# Autodesk Inventor assembly: Frame V2
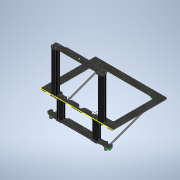
[picture p0: Inventor's stored thumbnail of the model, 180x180]
Saved by Autodesk Inventor 2020.3 (Build 243373010, 373A)
## iProperties
Created: 2019-06-17
Part Number: Frame V2
Document SubType Name: Assembly
Designer: pepd9
Author: pepd9
## Documents named in this file (13)
- D:\Designs\MK3PRO P1\FRAME\Frame V2.iam
- D:\Designs\MK3PRO P1\FRAME\FRONT PLATE P1.2.ipt
- D:\Designs\MK3PRO P1\FRAME\Long Extrusion.ipt
- D:\Designs\MK3PRO P1\COMPONENTS\90128A234_ZNC-PLTD ALLOY STL SCKT HEAD CAP SCREW.ipt
- D:\Designs\MK3PRO P1\FRAME\Short Extrusion.ipt
- D:\Designs\MK3PRO P1\FRAME\REAR PLATE P1.2.ipt
- D:\Designs\MK3PRO P1\FRAME\Angle Support Bottom Anchor.ipt
- D:\Designs\MK3PRO P1\FRAME\Angle Support Top Anchor.ipt
- D:\Designs\MK3PRO P1\COMPONENTS\WASHER_M10.ipt
- D:\Designs\MK3PRO P1\FRAME\Angle Support.ipt
- D:\Designs\MK3PRO P1\COMPONENTS\NUT_THIN_M10.ipt
- D:\Designs\MK3PRO P1\COMPONENTS\SHCS_M3_12.ipt
- D:\Designs\MK3PRO P1\FRAME\CENTER FRAME P2.0.ipt
## Components (85 placed, 12 different names)
1. CENTER FRAME P2.0:1 — Mate:1, Mate:2, Mate:3, Mate:4, Mate:5, Mate:6, Mate:7, Mate:8, Mate:9, Flush:1, Mate:23, Mate:24, Mate:25, Mate:28, Mate:37, Mate:38, Mate:39, Mate:40, Mate:41, Mate:42, Mate:43, Mate:44, Mate:45, Mate:46, Mate:47, Mate:48, Mate:49, Mate:50, Mate:51, Mate:52, Mate:53, Mate:54, Mate:55, Mate:56, Mate:57, Mate:58, Mate:59, Mate:60, Mate:61, Mate:62, Mate:63, Mate:64, Mate:65, Mate:66, Mate:96, Mate:97, Mate:98, Mate:99, Mate:100, Mate:101
2. Long Extrusion:1 — Mate:1, Mate:10, Mate:11, Mate:229
3. 90128A234_ZNC-PLTD ALLOY STL SCKT HEAD CAP SCREW:1 — Mate:2, Mate:3, Mate:10
4. 90128A234_ZNC-PLTD ALLOY STL SCKT HEAD CAP SCREW:2 — Mate:6, Mate:7
5. 90128A234_ZNC-PLTD ALLOY STL SCKT HEAD CAP SCREW:3 — Mate:5, Mate:8
6. 90128A234_ZNC-PLTD ALLOY STL SCKT HEAD CAP SCREW:4 — Mate:4, Mate:9, Mate:11
7. 90128A234_ZNC-PLTD ALLOY STL SCKT HEAD CAP SCREW:5 — Mate:231
8. 90128A234_ZNC-PLTD ALLOY STL SCKT HEAD CAP SCREW:6
9. 90128A234_ZNC-PLTD ALLOY STL SCKT HEAD CAP SCREW:7 — Mate:230
10. 90128A234_ZNC-PLTD ALLOY STL SCKT HEAD CAP SCREW:8
11. Long Extrusion:2 — Mate:25, Mate:28
12. 90128A234_ZNC-PLTD ALLOY STL SCKT HEAD CAP SCREW:9
13. 90128A234_ZNC-PLTD ALLOY STL SCKT HEAD CAP SCREW:10
14. 90128A234_ZNC-PLTD ALLOY STL SCKT HEAD CAP SCREW:11
15. 90128A234_ZNC-PLTD ALLOY STL SCKT HEAD CAP SCREW:12
16. 90128A234_ZNC-PLTD ALLOY STL SCKT HEAD CAP SCREW:13 — Mate:37, Mate:44
17. 90128A234_ZNC-PLTD ALLOY STL SCKT HEAD CAP SCREW:14 — Mate:38, Mate:42
18. 90128A234_ZNC-PLTD ALLOY STL SCKT HEAD CAP SCREW:15 — Mate:39, Mate:43
19. 90128A234_ZNC-PLTD ALLOY STL SCKT HEAD CAP SCREW:16 — Mate:40, Mate:41
20. Short Extrusion:1 — Mate:45, Mate:46, Mate:47
21. Short Extrusion:2 — Mate:48, Mate:49, Mate:50, Mate:67, Mate:68, Mate:69
22. 90128A234_ZNC-PLTD ALLOY STL SCKT HEAD CAP SCREW:17 — Mate:53, Mate:56
23. 90128A234_ZNC-PLTD ALLOY STL SCKT HEAD CAP SCREW:18 — Mate:54, Mate:58
24. 90128A234_ZNC-PLTD ALLOY STL SCKT HEAD CAP SCREW:19 — Mate:51, Mate:55
25. 90128A234_ZNC-PLTD ALLOY STL SCKT HEAD CAP SCREW:20 — Mate:52, Mate:57
26. 90128A234_ZNC-PLTD ALLOY STL SCKT HEAD CAP SCREW:21 — Mate:59, Mate:63
27. 90128A234_ZNC-PLTD ALLOY STL SCKT HEAD CAP SCREW:22 — Mate:60, Mate:64
28. 90128A234_ZNC-PLTD ALLOY STL SCKT HEAD CAP SCREW:23 — Mate:61, Mate:65
29. 90128A234_ZNC-PLTD ALLOY STL SCKT HEAD CAP SCREW:24 — Mate:62, Mate:66
30. REAR PLATE P1.2:1 — Mate:67, Mate:68, Mate:69, Mate:70, Mate:71, Mate:72, Mate:73, Mate:74, Mate:75, Mate:76, Mate:77, Mate:78, Mate:79, Mate:80, Mate:81, Mate:82, Mate:83, Mate:84, Mate:95, Mate:102, Mate:103
31. 90128A234_ZNC-PLTD ALLOY STL SCKT HEAD CAP SCREW:25 — Mate:70, Mate:83
32. 90128A234_ZNC-PLTD ALLOY STL SCKT HEAD CAP SCREW:26 — Mate:71, Mate:81
33. 90128A234_ZNC-PLTD ALLOY STL SCKT HEAD CAP SCREW:27 — Mate:73, Mate:84
34. 90128A234_ZNC-PLTD ALLOY STL SCKT HEAD CAP SCREW:28 — Mate:72, Mate:82
35. 90128A234_ZNC-PLTD ALLOY STL SCKT HEAD CAP SCREW:29 — Mate:76, Mate:78
36. 90128A234_ZNC-PLTD ALLOY STL SCKT HEAD CAP SCREW:30 — Mate:74, Mate:77
37. 90128A234_ZNC-PLTD ALLOY STL SCKT HEAD CAP SCREW:31 — Mate:75, Mate:79
38. 90128A234_ZNC-PLTD ALLOY STL SCKT HEAD CAP SCREW:32 — Mate:80, Mate:95
39. Angle Support Bottom Anchor:1 — Mate:102, Mate:104, Mate:106, Mate:107, Mate:108, Mate:109, Mate:168, Mate:169, Mate:170, Mate:171, Mate:172, Mate:173, Mate:174, Mate:175
40. Angle Support Bottom Anchor:2 — Mate:103, Mate:105, Mate:110, Mate:111, Mate:112, Mate:113, Mate:176, Mate:177, Mate:178, Mate:179, Mate:180, Mate:181, Mate:182, Mate:183
41. Angle Support Top Anchor:1 — Mate:96, Mate:98, Mate:99, Mate:104, Mate:114, Mate:115, Mate:116, Mate:117, Mate:122, Mate:156, Mate:157, Mate:158, Mate:159, Mate:184, Mate:185, Mate:186, Mate:187
42. Angle Support Top Anchor:2 — Mate:97, Mate:100, Mate:101, Mate:105, Mate:118, Mate:119, Mate:120, Mate:121, Mate:123, Mate:160, Mate:161, Mate:162, Mate:163, Mate:164, Mate:165, Mate:166, Mate:167
43. WASHER_M10:1 — Mate:116, Mate:117, Mate:138
44. WASHER_M10:2 — Mate:114, Mate:115, Mate:136
45. WASHER_M10:3 — Mate:119, Mate:120, Mate:130
46. WASHER_M10:4 — Mate:118, Mate:121, Mate:128
47. WASHER_M10:5 — Mate:110, Mate:111, Mate:149
48. WASHER_M10:6 — Mate:112, Mate:113, Mate:154
49. WASHER_M10:7 — Mate:106, Mate:107, Mate:141
50. WASHER_M10:8 — Mate:108, Mate:109, Mate:146
51. Angle Support:1 — Mate:122, Mate:132, Mate:133, Mate:134, Mate:135, Flush:2, Mate:140, Mate:142, Mate:144, Mate:145
52. Angle Support:2 — Mate:123, Mate:124, Mate:125, Mate:126, Mate:127, Flush:3, Mate:148, Mate:150, Mate:152, Mate:153
53. NUT_THIN_M10:1 — Mate:134, Mate:138, Mate:139
54. NUT_THIN_M10:2 — Mate:135, Mate:139
55. NUT_THIN_M10:3 — Mate:132, Mate:137, Flush:2
56. NUT_THIN_M10:4 — Mate:133, Mate:136, Mate:137
57. NUT_THIN_M10:5 — Mate:125, Mate:131, Flush:3
58. NUT_THIN_M10:6 — Mate:127, Mate:129
59. NUT_THIN_M10:7 — Mate:126, Mate:128, Mate:129
60. NUT_THIN_M10:8 — Mate:124, Mate:130, Mate:131
61. NUT_THIN_M10:9 — Mate:140, Mate:141, Mate:143
62. NUT_THIN_M10:10 — Mate:144, Mate:146, Mate:147
63. NUT_THIN_M10:11 — Mate:145, Mate:147
64. NUT_THIN_M10:12 — Mate:142, Mate:143
65. NUT_THIN_M10:13 — Mate:148, Mate:149, Mate:151
66. NUT_THIN_M10:14 — Mate:152, Mate:154, Mate:155
67. NUT_THIN_M10:15 — Mate:150, Mate:151
68. NUT_THIN_M10:16 — Mate:153, Mate:155, Flush:4
69. SHCS_M3_12:1 — Mate:171, Mate:175
70. SHCS_M3_12:2 — Mate:170, Mate:174
71. SHCS_M3_12:3 — Mate:169, Mate:172
72. SHCS_M3_12:4 — Mate:168, Mate:173
73. SHCS_M3_12:5 — Mate:179, Mate:180
74. SHCS_M3_12:6 — Mate:178, Mate:181
75. SHCS_M3_12:7 — Mate:177, Mate:183
76. SHCS_M3_12:8 — Mate:176, Mate:182
77. SHCS_M3_12:9 — Mate:156, Mate:184
78. SHCS_M3_12:10 — Mate:157, Mate:185
79. SHCS_M3_12:11 — Mate:158, Mate:186
80. SHCS_M3_12:12 — Mate:159, Mate:187
81. SHCS_M3_12:13 — Mate:163, Mate:167
82. SHCS_M3_12:14 — Mate:162, Mate:166
83. SHCS_M3_12:15 — Mate:161, Mate:165
84. SHCS_M3_12:16 — Mate:160, Mate:164
85. FRONT PLATE P1.2:1 — Mate:229, Mate:230, Mate:231
## Relationships (163: Mate 159, Flush 4)
- Mate:1: CENTER FRAME P2.0:1 ↔ Long Extrusion:1
- Mate:2: CENTER FRAME P2.0:1 ↔ 90128A234_ZNC-PLTD ALLOY STL SCKT HEAD CAP SCREW:1
- Mate:3: CENTER FRAME P2.0:1 ↔ 90128A234_ZNC-PLTD ALLOY STL SCKT HEAD CAP SCREW:1
- Mate:4: CENTER FRAME P2.0:1 ↔ 90128A234_ZNC-PLTD ALLOY STL SCKT HEAD CAP SCREW:4
- Mate:5: CENTER FRAME P2.0:1 ↔ 90128A234_ZNC-PLTD ALLOY STL SCKT HEAD CAP SCREW:3
- Mate:6: CENTER FRAME P2.0:1 ↔ 90128A234_ZNC-PLTD ALLOY STL SCKT HEAD CAP SCREW:2
- Mate:7: CENTER FRAME P2.0:1 ↔ 90128A234_ZNC-PLTD ALLOY STL SCKT HEAD CAP SCREW:2
- Mate:8: CENTER FRAME P2.0:1 ↔ 90128A234_ZNC-PLTD ALLOY STL SCKT HEAD CAP SCREW:3
- Mate:9: CENTER FRAME P2.0:1 ↔ 90128A234_ZNC-PLTD ALLOY STL SCKT HEAD CAP SCREW:4
- Mate:10: Long Extrusion:1 ↔ 90128A234_ZNC-PLTD ALLOY STL SCKT HEAD CAP SCREW:1
- Mate:11: Long Extrusion:1 ↔ 90128A234_ZNC-PLTD ALLOY STL SCKT HEAD CAP SCREW:4
- Flush:1 (-245 mm): CENTER FRAME P2.0:1
- Mate:23: CENTER FRAME P2.0:1
- Mate:24 (-24.5 mm): CENTER FRAME P2.0:1
- Mate:25: CENTER FRAME P2.0:1 ↔ Long Extrusion:2
- Mate:28: CENTER FRAME P2.0:1 ↔ Long Extrusion:2
- Mate:37: CENTER FRAME P2.0:1 ↔ 90128A234_ZNC-PLTD ALLOY STL SCKT HEAD CAP SCREW:13
- Mate:38: CENTER FRAME P2.0:1 ↔ 90128A234_ZNC-PLTD ALLOY STL SCKT HEAD CAP SCREW:14
- Mate:39: CENTER FRAME P2.0:1 ↔ 90128A234_ZNC-PLTD ALLOY STL SCKT HEAD CAP SCREW:15
- Mate:40: CENTER FRAME P2.0:1 ↔ 90128A234_ZNC-PLTD ALLOY STL SCKT HEAD CAP SCREW:16
- Mate:41: CENTER FRAME P2.0:1 ↔ 90128A234_ZNC-PLTD ALLOY STL SCKT HEAD CAP SCREW:16
- Mate:42: CENTER FRAME P2.0:1 ↔ 90128A234_ZNC-PLTD ALLOY STL SCKT HEAD CAP SCREW:14
- Mate:43: CENTER FRAME P2.0:1 ↔ 90128A234_ZNC-PLTD ALLOY STL SCKT HEAD CAP SCREW:15
- Mate:44: CENTER FRAME P2.0:1 ↔ 90128A234_ZNC-PLTD ALLOY STL SCKT HEAD CAP SCREW:13
- Mate:45: CENTER FRAME P2.0:1 ↔ Short Extrusion:1
- Mate:46: CENTER FRAME P2.0:1 ↔ Short Extrusion:1
- Mate:47: CENTER FRAME P2.0:1 ↔ Short Extrusion:1
- Mate:48: CENTER FRAME P2.0:1 ↔ Short Extrusion:2
- Mate:49: CENTER FRAME P2.0:1 ↔ Short Extrusion:2
- Mate:50: CENTER FRAME P2.0:1 ↔ Short Extrusion:2
- Mate:51: CENTER FRAME P2.0:1 ↔ 90128A234_ZNC-PLTD ALLOY STL SCKT HEAD CAP SCREW:19
- Mate:52: CENTER FRAME P2.0:1 ↔ 90128A234_ZNC-PLTD ALLOY STL SCKT HEAD CAP SCREW:20
- Mate:53: CENTER FRAME P2.0:1 ↔ 90128A234_ZNC-PLTD ALLOY STL SCKT HEAD CAP SCREW:17
- Mate:54: CENTER FRAME P2.0:1 ↔ 90128A234_ZNC-PLTD ALLOY STL SCKT HEAD CAP SCREW:18
- Mate:55: CENTER FRAME P2.0:1 ↔ 90128A234_ZNC-PLTD ALLOY STL SCKT HEAD CAP SCREW:19
- Mate:56: CENTER FRAME P2.0:1 ↔ 90128A234_ZNC-PLTD ALLOY STL SCKT HEAD CAP SCREW:17
- Mate:57: CENTER FRAME P2.0:1 ↔ 90128A234_ZNC-PLTD ALLOY STL SCKT HEAD CAP SCREW:20
- Mate:58: CENTER FRAME P2.0:1 ↔ 90128A234_ZNC-PLTD ALLOY STL SCKT HEAD CAP SCREW:18
- Mate:59: CENTER FRAME P2.0:1 ↔ 90128A234_ZNC-PLTD ALLOY STL SCKT HEAD CAP SCREW:21
- Mate:60: CENTER FRAME P2.0:1 ↔ 90128A234_ZNC-PLTD ALLOY STL SCKT HEAD CAP SCREW:22
- Mate:61: CENTER FRAME P2.0:1 ↔ 90128A234_ZNC-PLTD ALLOY STL SCKT HEAD CAP SCREW:23
- Mate:62: CENTER FRAME P2.0:1 ↔ 90128A234_ZNC-PLTD ALLOY STL SCKT HEAD CAP SCREW:24
- Mate:63: CENTER FRAME P2.0:1 ↔ 90128A234_ZNC-PLTD ALLOY STL SCKT HEAD CAP SCREW:21
- Mate:64: CENTER FRAME P2.0:1 ↔ 90128A234_ZNC-PLTD ALLOY STL SCKT HEAD CAP SCREW:22
- Mate:65: CENTER FRAME P2.0:1 ↔ 90128A234_ZNC-PLTD ALLOY STL SCKT HEAD CAP SCREW:23
- Mate:66: CENTER FRAME P2.0:1 ↔ 90128A234_ZNC-PLTD ALLOY STL SCKT HEAD CAP SCREW:24
- Mate:67: Short Extrusion:2 ↔ REAR PLATE P1.2:1
- Mate:68: Short Extrusion:2 ↔ REAR PLATE P1.2:1
- Mate:69: Short Extrusion:2 ↔ REAR PLATE P1.2:1
- Mate:70: REAR PLATE P1.2:1 ↔ 90128A234_ZNC-PLTD ALLOY STL SCKT HEAD CAP SCREW:25
- Mate:71: REAR PLATE P1.2:1 ↔ 90128A234_ZNC-PLTD ALLOY STL SCKT HEAD CAP SCREW:26
- Mate:72: REAR PLATE P1.2:1 ↔ 90128A234_ZNC-PLTD ALLOY STL SCKT HEAD CAP SCREW:28
- Mate:73: REAR PLATE P1.2:1 ↔ 90128A234_ZNC-PLTD ALLOY STL SCKT HEAD CAP SCREW:27
- Mate:74: REAR PLATE P1.2:1 ↔ 90128A234_ZNC-PLTD ALLOY STL SCKT HEAD CAP SCREW:30
- Mate:75: REAR PLATE P1.2:1 ↔ 90128A234_ZNC-PLTD ALLOY STL SCKT HEAD CAP SCREW:31
- Mate:76: REAR PLATE P1.2:1 ↔ 90128A234_ZNC-PLTD ALLOY STL SCKT HEAD CAP SCREW:29
- Mate:77: REAR PLATE P1.2:1 ↔ 90128A234_ZNC-PLTD ALLOY STL SCKT HEAD CAP SCREW:30
- Mate:78: REAR PLATE P1.2:1 ↔ 90128A234_ZNC-PLTD ALLOY STL SCKT HEAD CAP SCREW:29
- Mate:79: REAR PLATE P1.2:1 ↔ 90128A234_ZNC-PLTD ALLOY STL SCKT HEAD CAP SCREW:31
- Mate:80: REAR PLATE P1.2:1 ↔ 90128A234_ZNC-PLTD ALLOY STL SCKT HEAD CAP SCREW:32
- Mate:81: REAR PLATE P1.2:1 ↔ 90128A234_ZNC-PLTD ALLOY STL SCKT HEAD CAP SCREW:26
- Mate:82: REAR PLATE P1.2:1 ↔ 90128A234_ZNC-PLTD ALLOY STL SCKT HEAD CAP SCREW:28
- Mate:83: REAR PLATE P1.2:1 ↔ 90128A234_ZNC-PLTD ALLOY STL SCKT HEAD CAP SCREW:25
- Mate:84: REAR PLATE P1.2:1 ↔ 90128A234_ZNC-PLTD ALLOY STL SCKT HEAD CAP SCREW:27
- Mate:95: REAR PLATE P1.2:1 ↔ 90128A234_ZNC-PLTD ALLOY STL SCKT HEAD CAP SCREW:32
- Mate:96: CENTER FRAME P2.0:1 ↔ Angle Support Top Anchor:1
- Mate:97: CENTER FRAME P2.0:1 ↔ Angle Support Top Anchor:2
- Mate:98: CENTER FRAME P2.0:1 ↔ Angle Support Top Anchor:1
- Mate:99: CENTER FRAME P2.0:1 ↔ Angle Support Top Anchor:1
- Mate:100: CENTER FRAME P2.0:1 ↔ Angle Support Top Anchor:2
- Mate:101: CENTER FRAME P2.0:1 ↔ Angle Support Top Anchor:2
- Mate:102: REAR PLATE P1.2:1 ↔ Angle Support Bottom Anchor:1
- Mate:103: REAR PLATE P1.2:1 ↔ Angle Support Bottom Anchor:2
- Mate:104: Angle Support Bottom Anchor:1 ↔ Angle Support Top Anchor:1
- Mate:105: Angle Support Bottom Anchor:2 ↔ Angle Support Top Anchor:2
- Mate:106: Angle Support Bottom Anchor:1 ↔ WASHER_M10:7
- Mate:107: Angle Support Bottom Anchor:1 ↔ WASHER_M10:7
- Mate:108: Angle Support Bottom Anchor:1 ↔ WASHER_M10:8
- Mate:109: Angle Support Bottom Anchor:1 ↔ WASHER_M10:8
- Mate:110: Angle Support Bottom Anchor:2 ↔ WASHER_M10:5
- Mate:111: Angle Support Bottom Anchor:2 ↔ WASHER_M10:5
- Mate:112: Angle Support Bottom Anchor:2 ↔ WASHER_M10:6
- Mate:113: Angle Support Bottom Anchor:2 ↔ WASHER_M10:6
- Mate:114: Angle Support Top Anchor:1 ↔ WASHER_M10:2
- Mate:115: Angle Support Top Anchor:1 ↔ WASHER_M10:2
- Mate:116: Angle Support Top Anchor:1 ↔ WASHER_M10:1
- Mate:117: Angle Support Top Anchor:1 ↔ WASHER_M10:1
- Mate:118: Angle Support Top Anchor:2 ↔ WASHER_M10:4
- Mate:119: Angle Support Top Anchor:2 ↔ WASHER_M10:3
- Mate:120: Angle Support Top Anchor:2 ↔ WASHER_M10:3
- Mate:121: Angle Support Top Anchor:2 ↔ WASHER_M10:4
- Mate:122: Angle Support Top Anchor:1 ↔ Angle Support:1
- Mate:123: Angle Support Top Anchor:2 ↔ Angle Support:2
- Mate:124: Angle Support:2 ↔ NUT_THIN_M10:8
- Mate:125: Angle Support:2 ↔ NUT_THIN_M10:5
- Mate:126: Angle Support:2 ↔ NUT_THIN_M10:7
- Mate:127: Angle Support:2 ↔ NUT_THIN_M10:6
- Mate:128: WASHER_M10:4 ↔ NUT_THIN_M10:7
- Mate:129: NUT_THIN_M10:6 ↔ NUT_THIN_M10:7
- Mate:130: WASHER_M10:3 ↔ NUT_THIN_M10:8
- Mate:131: NUT_THIN_M10:5 ↔ NUT_THIN_M10:8
- Mate:132: Angle Support:1 ↔ NUT_THIN_M10:3
- Mate:133: Angle Support:1 ↔ NUT_THIN_M10:4
- Mate:134: Angle Support:1 ↔ NUT_THIN_M10:1
- Mate:135: Angle Support:1 ↔ NUT_THIN_M10:2
- Mate:136: WASHER_M10:2 ↔ NUT_THIN_M10:4
- Mate:137: NUT_THIN_M10:3 ↔ NUT_THIN_M10:4
- Mate:138: WASHER_M10:1 ↔ NUT_THIN_M10:1
- Mate:139: NUT_THIN_M10:1 ↔ NUT_THIN_M10:2
- Flush:2 (5 mm): Angle Support:1 ↔ NUT_THIN_M10:3
- Flush:3 (5 mm): Angle Support:2 ↔ NUT_THIN_M10:5
- Mate:140: Angle Support:1 ↔ NUT_THIN_M10:9
- Mate:141: WASHER_M10:7 ↔ NUT_THIN_M10:9
- Mate:142: Angle Support:1 ↔ NUT_THIN_M10:12
- Mate:143: NUT_THIN_M10:9 ↔ NUT_THIN_M10:12
- Mate:144: Angle Support:1 ↔ NUT_THIN_M10:10
- Mate:145: Angle Support:1 ↔ NUT_THIN_M10:11
- Mate:146: WASHER_M10:8 ↔ NUT_THIN_M10:10
- Mate:147: NUT_THIN_M10:10 ↔ NUT_THIN_M10:11
- Mate:148: Angle Support:2 ↔ NUT_THIN_M10:13
- Mate:149: WASHER_M10:5 ↔ NUT_THIN_M10:13
- Mate:150: Angle Support:2 ↔ NUT_THIN_M10:15
- Mate:151: NUT_THIN_M10:13 ↔ NUT_THIN_M10:15
- Mate:152: Angle Support:2 ↔ NUT_THIN_M10:14
- Mate:153: Angle Support:2 ↔ NUT_THIN_M10:16
- Mate:154: WASHER_M10:6 ↔ NUT_THIN_M10:14
- Mate:155: NUT_THIN_M10:14 ↔ NUT_THIN_M10:16
- Mate:156: Angle Support Top Anchor:1 ↔ SHCS_M3_12:9
- Mate:157: Angle Support Top Anchor:1 ↔ SHCS_M3_12:10
- Mate:158: Angle Support Top Anchor:1 ↔ SHCS_M3_12:11
- Mate:159: Angle Support Top Anchor:1 ↔ SHCS_M3_12:12
- Mate:160: Angle Support Top Anchor:2 ↔ SHCS_M3_12:16
- Mate:161: Angle Support Top Anchor:2 ↔ SHCS_M3_12:15
- Mate:162: Angle Support Top Anchor:2 ↔ SHCS_M3_12:14
- Mate:163: Angle Support Top Anchor:2 ↔ SHCS_M3_12:13
- Mate:164: Angle Support Top Anchor:2 ↔ SHCS_M3_12:16
- Mate:165: Angle Support Top Anchor:2 ↔ SHCS_M3_12:15
- Mate:166: Angle Support Top Anchor:2 ↔ SHCS_M3_12:14
- Mate:167: Angle Support Top Anchor:2 ↔ SHCS_M3_12:13
- Mate:168: Angle Support Bottom Anchor:1 ↔ SHCS_M3_12:4
- Mate:169: Angle Support Bottom Anchor:1 ↔ SHCS_M3_12:3
- Mate:170: Angle Support Bottom Anchor:1 ↔ SHCS_M3_12:2
- Mate:171: Angle Support Bottom Anchor:1 ↔ SHCS_M3_12:1
- Mate:172: Angle Support Bottom Anchor:1 ↔ SHCS_M3_12:3
- Mate:173: Angle Support Bottom Anchor:1 ↔ SHCS_M3_12:4
- Mate:174: Angle Support Bottom Anchor:1 ↔ SHCS_M3_12:2
- Mate:175: Angle Support Bottom Anchor:1 ↔ SHCS_M3_12:1
- Mate:176: Angle Support Bottom Anchor:2 ↔ SHCS_M3_12:8
- Mate:177: Angle Support Bottom Anchor:2 ↔ SHCS_M3_12:7
- Mate:178: Angle Support Bottom Anchor:2 ↔ SHCS_M3_12:6
- Mate:179: Angle Support Bottom Anchor:2 ↔ SHCS_M3_12:5
- Mate:180: Angle Support Bottom Anchor:2 ↔ SHCS_M3_12:5
- Mate:181: Angle Support Bottom Anchor:2 ↔ SHCS_M3_12:6
- Mate:182: Angle Support Bottom Anchor:2 ↔ SHCS_M3_12:8
- Mate:183: Angle Support Bottom Anchor:2 ↔ SHCS_M3_12:7
- Mate:184: Angle Support Top Anchor:1 ↔ SHCS_M3_12:9
- Mate:185: Angle Support Top Anchor:1 ↔ SHCS_M3_12:10
- Mate:186: Angle Support Top Anchor:1 ↔ SHCS_M3_12:11
- Mate:187: Angle Support Top Anchor:1 ↔ SHCS_M3_12:12
- Flush:4 (40 mm): NUT_THIN_M10:16
- Mate:229: Long Extrusion:1 ↔ FRONT PLATE P1.2:1
- Mate:230: 90128A234_ZNC-PLTD ALLOY STL SCKT HEAD CAP SCREW:7 ↔ FRONT PLATE P1.2:1
- Mate:231: 90128A234_ZNC-PLTD ALLOY STL SCKT HEAD CAP SCREW:5 ↔ FRONT PLATE P1.2:1
